# Autodesk Inventor assembly: leg_flame_assy
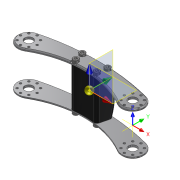
[picture p0: Inventor's stored thumbnail of the model, 180x180]
Saved by Autodesk Inventor 2019.4 (Build 234330000, 330)
## iProperties
Created: 2018-08-12
Part Number: leg_flame_assy
Material: 一般
Document SubType Name: Assembly
Designer: y6tada
Mass: 42.9223 g
Surface Area: 147.897 cm^2
Volume: 24.3475 cm^3
Density: 1.7629 g/cm^3
Author: y6tada
## Documents named in this file (5)
- C:\Workspace\HaptHexa\Hardware\Inventor\Femur\_Femur.iam
- C:\Workspace\HaptHexa\Hardware\Inventor\Femur\spacer.ipt
- C:\Workspace\HaptHexa\Hardware\Inventor\Femur\side_frame.ipt
- C:\Workspace\HaptHexa\Hardware\Inventor\Femur\side_frame_mir.ipt
- C:\Users\y6tada\Documents\Inventor\Content Center Files\R2019\ja-JP\JIS B 1176\JIS B 1176 - M3 x 6 - 0.5.ipt
## Components (11 placed, 4 different names)
1. leg_spacer — メイト:1, フラッシュ:3, フラッシュ:4, メイト:7, メイト:8, メイト:9, メイト:11
2. side_frame:1 — メイト:1, メイト:6, フラッシュ:3, フラッシュ:4, 挿入:5, 挿入:6, 挿入:7, 挿入:8, メイト:10, フラッシュ:5
3. side_frame_mir:1 — メイト:7, メイト:8, メイト:9, 挿入:1, 挿入:2, 挿入:3, 挿入:4
4. JIS B 1176 - メートル M3 x 6:1 — 挿入:1
5. JIS B 1176 - メートル M3 x 6:2 — 挿入:2
6. JIS B 1176 - メートル M3 x 6:3 — 挿入:3
7. JIS B 1176 - メートル M3 x 6:4 — 挿入:4
8. JIS B 1176 - メートル M3 x 6:5 — 挿入:5
9. JIS B 1176 - メートル M3 x 6:6 — 挿入:6
10. JIS B 1176 - メートル M3 x 6:7 — 挿入:7
11. JIS B 1176 - メートル M3 x 6:8 — 挿入:8
## Relationships (18: Insert 8, Mate 7, Flush 3)
- メイト:1 [Mate]: leg_spacer ↔ side_frame:1
- メイト:6 [Mate]: side_frame:1
- フラッシュ:3 [Flush]: leg_spacer ↔ side_frame:1
- フラッシュ:4 [Flush]: leg_spacer ↔ side_frame:1
- メイト:7 [Mate]: leg_spacer ↔ side_frame_mir:1
- メイト:8 [Mate]: leg_spacer ↔ side_frame_mir:1
- メイト:9 [Mate]: leg_spacer ↔ side_frame_mir:1
- 挿入:1 [Insert]: side_frame_mir:1 ↔ JIS B 1176 - メートル M3 x 6:1
- 挿入:2 [Insert]: side_frame_mir:1 ↔ JIS B 1176 - メートル M3 x 6:2
- 挿入:3 [Insert]: side_frame_mir:1 ↔ JIS B 1176 - メートル M3 x 6:3
- 挿入:4 [Insert]: side_frame_mir:1 ↔ JIS B 1176 - メートル M3 x 6:4
- 挿入:5 [Insert]: side_frame:1 ↔ JIS B 1176 - メートル M3 x 6:5
- 挿入:6 [Insert]: side_frame:1 ↔ JIS B 1176 - メートル M3 x 6:6
- 挿入:7 [Insert]: side_frame:1 ↔ JIS B 1176 - メートル M3 x 6:7
- 挿入:8 [Insert]: side_frame:1 ↔ JIS B 1176 - メートル M3 x 6:8
- メイト:10 [Mate]: side_frame:1
- フラッシュ:5 [Flush]: side_frame:1
- メイト:11 [Mate]: leg_spacer
